# Autodesk Inventor assembly: LegBaseUnitBasis
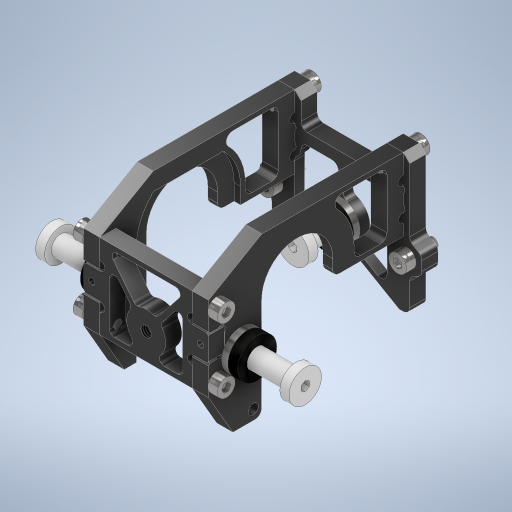
[picture p0: Inventor's stored thumbnail of the model, 512x512]
Saved by Autodesk Inventor 2024.2 (Build 282272000, 272)
## iProperties
Created: 2024-01-08
Part Number: LegBaseUnitBasis
Document SubType Name: Assembly
Designer: Masato Kubotera
Mass: 71.6116 g
Surface Area: 191.118 cm^2
Volume: 19.3216 cm^3
Density: 3.70629 g/cm^3
Author: Masato Kubotera
## Documents named in this file (11)
- C:\Users\masato\OneDrive - Chiba Institute of Technology\CIT Brains\RoboCup2024\Mechanic\SUSTAINA-OP2\NativeFiles\Boby\LowerLimb\Legs\LegBases\LegBaseUnitBasis.iam
- C:\Users\masato\OneDrive - Chiba Institute of Technology\CIT Brains\RoboCup2024\Mechanic\SUSTAINA-OP2\NativeFiles\Boby\COTS\Washers\Resin\CC-0612-30B.ipt
- C:\Users\masato\OneDrive - Chiba Institute of Technology\CIT Brains\RoboCup2024\Mechanic\SUSTAINA-OP2\NativeFiles\Boby\COTS\Washers\Metal\UUW-0412-20H.ipt
- C:\Users\masato\OneDrive - Chiba Institute of Technology\CIT Brains\RoboCup2024\Mechanic\SUSTAINA-OP2\NativeFiles\Boby\COTS\Screws\ScrewsWithShoulder\DBTSY4-15-5-DHC.ipt
- C:\Users\masato\OneDrive - Chiba Institute of Technology\CIT Brains\RoboCup2024\Mechanic\SUSTAINA-OP2\NativeFiles\Boby\COTS\Screws\CapScrew\UC-0308.ipt
- C:\Users\masato\OneDrive - Chiba Institute of Technology\CIT Brains\RoboCup2024\Mechanic\SUSTAINA-OP2\NativeFiles\Boby\LowerLimb\Legs\LegBases\LegBaseBackFulcrumFrame.ipt
- C:\Users\masato\OneDrive - Chiba Institute of Technology\CIT Brains\RoboCup2024\Mechanic\SUSTAINA-OP2\NativeFiles\Boby\LowerLimb\Legs\LegBases\LegBaseSideFrame.ipt
- C:\Users\masato\OneDrive - Chiba Institute of Technology\CIT Brains\RoboCup2024\Mechanic\SUSTAINA-OP2\NativeFiles\Boby\LowerLimb\Legs\LegBases\LegBaseSideFrame_MIR.ipt
- C:\Users\masato\OneDrive - Chiba Institute of Technology\CIT Brains\RoboCup2024\Mechanic\SUSTAINA-OP2\NativeFiles\Boby\LowerLimb\Legs\LegBases\LegBaseFrontFulcrumFrame.ipt
- C:\Users\masato\OneDrive - Chiba Institute of Technology\CIT Brains\RoboCup2024\Mechanic\SUSTAINA-OP2\NativeFiles\Boby\COTS\Screws\ScrewsWithShoulder\DBTSY4-10-5-DHC.ipt
- C:\Users\masato\OneDrive - Chiba Institute of Technology\CIT Brains\RoboCup2024\Mechanic\SUSTAINA-OP2\NativeFiles\Boby\COTS\Screws\CapScrew\UC-0310.ipt
## Components (21 placed, 10 different names)
1. LegBaseBackFulcrumFrame:1 — Flush:3, Insert:13, Insert:41, Insert:42, Insert:43, Insert:44, Insert:45, Insert:46
2. LegBaseSideFrame:1 — Flush:1, Flush:2, Insert:28, Insert:32, Insert:34, Insert:41
3. LegBaseSideFrame_MIR:1 — Mate:1, Angle:1, Flush:1, Flush:2, Insert:1, Insert:25, Insert:31, Insert:33, Insert:42
4. LegBaseFrontFulcrumFrame:1 — Insert:1, Angle:2
5. UC-0308:9 — Insert:43
6. UC-0308:10 — Insert:44
7. UC-0310:1 — Insert:45
8. UC-0310:2 — Insert:46
9. UC-0308:1 — Insert:31
10. UC-0308:3 — Insert:32
11. UC-0308:5 — Insert:33
12. UC-0308:6 — Insert:34
13. CC-0612-30B:1 — Insert:14
14. UUW-0412-20H:1 — Insert:13, Insert:14, Insert:15
15. UUW-0412-20H:2 — Insert:25, Insert:26, Insert:27
16. UUW-0412-20H:3 — Insert:28, Insert:29, Insert:30
17. CC-0612-30B:2 — Insert:26
18. CC-0612-30B:3 — Insert:29
19. DBTSY4-15-5-DHC:1 — Insert:27
20. DBTSY4-15-5-DHC:2 — Insert:30
21. DBTSY4-10-5-DHC:1 — Insert:15
## Relationships (26: Insert 20, Flush 3, Angle 2, Mate 1)
- Mate:1: LegBaseSideFrame_MIR:1
- Angle:1 (0 deg): LegBaseSideFrame_MIR:1
- Flush:1: LegBaseSideFrame:1 ↔ LegBaseSideFrame_MIR:1
- Flush:2: LegBaseSideFrame:1 ↔ LegBaseSideFrame_MIR:1
- Flush:3: LegBaseBackFulcrumFrame:1
- Insert:1: LegBaseSideFrame_MIR:1 ↔ LegBaseFrontFulcrumFrame:1
- Insert:13: LegBaseBackFulcrumFrame:1 ↔ UUW-0412-20H:1
- Insert:14: CC-0612-30B:1 ↔ UUW-0412-20H:1
- Insert:15: UUW-0412-20H:1 ↔ DBTSY4-10-5-DHC:1
- Insert:25: LegBaseSideFrame_MIR:1 ↔ UUW-0412-20H:2
- Insert:26: UUW-0412-20H:2 ↔ CC-0612-30B:2
- Insert:27: UUW-0412-20H:2 ↔ DBTSY4-15-5-DHC:1
- Insert:28: LegBaseSideFrame:1 ↔ UUW-0412-20H:3
- Insert:29: UUW-0412-20H:3 ↔ CC-0612-30B:3
- Insert:30: UUW-0412-20H:3 ↔ DBTSY4-15-5-DHC:2
- Insert:31: LegBaseSideFrame_MIR:1 ↔ UC-0308:1
- Insert:32: LegBaseSideFrame:1 ↔ UC-0308:3
- Insert:33: LegBaseSideFrame_MIR:1 ↔ UC-0308:5
- Insert:34: LegBaseSideFrame:1 ↔ UC-0308:6
- Angle:2 (180 deg): LegBaseFrontFulcrumFrame:1
- Insert:41: LegBaseBackFulcrumFrame:1 ↔ LegBaseSideFrame:1
- Insert:42: LegBaseBackFulcrumFrame:1 ↔ LegBaseSideFrame_MIR:1
- Insert:43: LegBaseBackFulcrumFrame:1 ↔ UC-0308:9
- Insert:44: LegBaseBackFulcrumFrame:1 ↔ UC-0308:10
- Insert:45: LegBaseBackFulcrumFrame:1 ↔ UC-0310:1
- Insert:46: LegBaseBackFulcrumFrame:1 ↔ UC-0310:2
